# Autodesk Inventor assembly: back_plates_MIR1
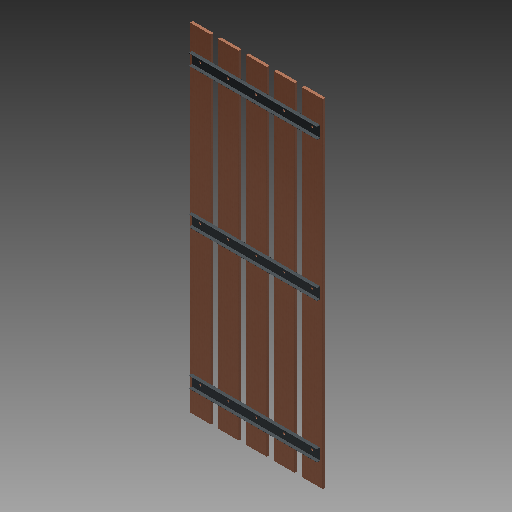
[picture p0: Inventor's stored thumbnail of the model, 512x512]
Saved by Autodesk Inventor 2019 (Build 230136000, 136)
## iProperties
Created: 2019-02-23
Part Number: back_plates_MIR1
Document SubType Name: Assembly
Designer: gaincarlo
Author: gaincarlo
## Documents named in this file (3)
- D:\Giancarlo Bacchio\Documenti\00 - Progetti\30-Inventor\LaPanca\back_plates_MIR1.iam
- D:\Giancarlo Bacchio\Documenti\00 - Progetti\30-Inventor\LaPanca\support1_MIR2.ipt
- D:\Giancarlo Bacchio\Documenti\00 - Progetti\30-Inventor\LaPanca\doga_long1_MIR4.ipt
## Components (8 placed, 2 different names)
1. support1_MIR2:1 — Mate:2, Mate:1, Mate:7
2. support1_MIR2:2 — Mate:5, Mate:3, Mate:9
3. support1_MIR2:3 — Mate:6, Mate:4, Mate:8
4. doga_long1_MIR4:1 — Mate:6, Mate:5, Mate:4, Mate:3, Mate:2, Mate:1
5. doga_long1_MIR4:2
6. doga_long1_MIR4:3 — Mate:9, Mate:8, Mate:7
7. doga_long1_MIR4:4
8. doga_long1_MIR4:5
## Component patterns: (5 elements, first: doga_long1_MIR4:1)
## Relationships (9: Mate 9)
- Mate:6: support1_MIR2:3 ↔ doga_long1_MIR4:1
- Mate:5: support1_MIR2:2 ↔ doga_long1_MIR4:1
- Mate:4: support1_MIR2:3 ↔ doga_long1_MIR4:1
- Mate:3: support1_MIR2:2 ↔ doga_long1_MIR4:1
- Mate:2: support1_MIR2:1 ↔ doga_long1_MIR4:1
- Mate:1: support1_MIR2:1 ↔ doga_long1_MIR4:1
- Mate:9: support1_MIR2:2 ↔ doga_long1_MIR4:3
- Mate:8: support1_MIR2:3 ↔ doga_long1_MIR4:3
- Mate:7: support1_MIR2:1 ↔ doga_long1_MIR4:3
